# Autodesk Inventor assembly: whole car
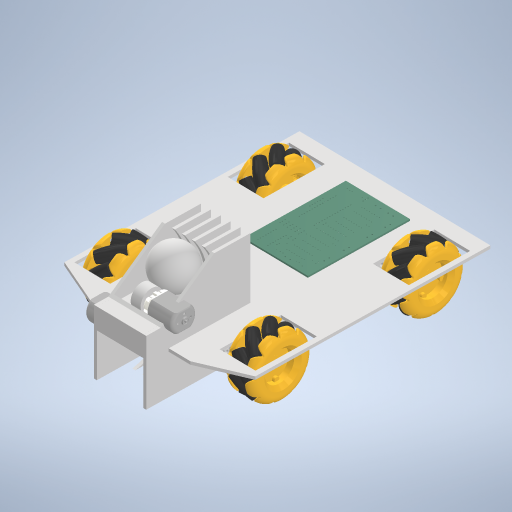
[picture p0: Inventor's stored thumbnail of the model, 512x512]
Saved by Autodesk Inventor 2023.2 (Build 272271030, 271C)
## iProperties
Created: 2023-06-19
Part Number: whole car
Document SubType Name: Assembly
Designer: kao91
Author: kao91
## Documents named in this file (16)
- C:\Users\kao91\Desktop\github\NTNU_mechatronic_practice_project\car design\whole car.iam
- C:\Users\kao91\Desktop\github\NTNU_mechatronic_practice_project\car design\DC Motor Gearbox\DC Motor Gearbox.ipt
- C:\Users\kao91\Desktop\github\NTNU_mechatronic_practice_project\car design\DC Motor Gearbox\DC Motor Gearbox_MIR.ipt
- C:\Users\kao91\Desktop\github\NTNU_mechatronic_practice_project\car design\df-robot-48mm-mecanum-wheel-left-side-1.snapshot.2\Mecanum Left v5\Mecanum Ra.ipt
- C:\Users\kao91\Desktop\github\NTNU_mechatronic_practice_project\car design\motor_to_mecanum_connector.ipt
- C:\Users\kao91\Desktop\github\NTNU_mechatronic_practice_project\car design\floor.ipt
- C:\Users\kao91\Desktop\github\NTNU_mechatronic_practice_project\car design\car platform.ipt
- C:\Users\kao91\Desktop\github\NTNU_mechatronic_practice_project\car design\df-robot-48mm-mecanum-wheel-left-side-1.snapshot.2\Mecanum Left v5\Mecanum Rb.ipt
- C:\Users\kao91\Desktop\github\NTNU_mechatronic_practice_project\car design\circuitPCB\circuitPCB.ipt
- C:\Users\kao91\Desktop\github\NTNU_mechatronic_practice_project\car design\collectballLR.ipt
- C:\Users\kao91\Desktop\github\NTNU_mechatronic_practice_project\car design\lr.ipt
- C:\Users\kao91\Desktop\github\NTNU_mechatronic_practice_project\car design\PING pong.ipt
- C:\Users\kao91\Desktop\github\NTNU_mechatronic_practice_project\car design\ROTATE.ipt
- C:\Users\kao91\Desktop\github\NTNU_mechatronic_practice_project\car design\FC-280PT-20150 12V DC Motor v3\FC-280PT-20150 12V DC Motor v3.ipt
- C:\Users\kao91\Desktop\github\NTNU_mechatronic_practice_project\car design\roll.ipt
- C:\Users\kao91\Desktop\github\NTNU_mechatronic_practice_project\car design\shoot.ipt
## Components (27 placed, 15 different names)
1. floor:1 — Mate:5, Tangent:5, Mate:23, Mate:24
2. car platform:1 — Flush:9, Mate:6, Mate:8, Mate:11, Mate:12, Mate:13, Mate:14, Mate:15, Mate:16, Flush:17, Flush:18, Flush:19, Flush:20, Mate:17, Flush:21, Mate:18, Mate:19, Mate:20, Mate:21, Mate:22
3. circuitPCB:1 — Mate:6, Flush:19
4. collectballLR:1 — Mate:15, Flush:16, Mate:16
5. collectballLR:2 — Mate:8, Mate:11, Flush:12, Flush:13, Flush:16, Tangent:2
6. collectballLR:3 — Flush:12, Flush:13, Flush:14, Flush:15, Mate:14, Tangent:3
7. collectballLR:4 — Mate:12, Flush:14, Flush:15, Mate:13, Mate:17
8. lr:1 — Flush:21, Mate:18, Mate:19, Tangent:4, Flush:22, Flush:23, Flush:25
9. lr:2 — Mate:20, Mate:21, Mate:22, Flush:24
10. PING pong:1 — Tangent:2, Tangent:3, Tangent:4
11. ROTATE:1 — Flush:22, Mate:25, Flush:23, Flush:24, Flush:27, Flush:28
12. FC-280PT-20150 12V DC Motor v3:1 — Flush:27, Flush:28, Rotational:12
13. FC-280PT-20150 12V DC Motor v3:2 — Mate:25, Flush:25, Flush:26, Rigid:1
14. roll:1 — Flush:26, Rigid:1
15. shoot:1 — Rotational:12
16. DC Motor Gearbox:1 — Rotational:1, Flush:1, Flush:6, Flush:7
17. Mecanum Ra:2 — Rotational:8, Mate:5
18. motor_to_mecanum_connector:1 — Rotational:1, Rotational:8
19. DC Motor Gearbox_MIR:1 — Rotational:4, Flush:2, Flush:5, Flush:7, Flush:17, Flush:20
20. motor_to_mecanum_connector:2 — Rotational:4, Rotational:10, Mate:23
21. Mecanum Rb:2 — Rotational:10
22. DC Motor Gearbox:2 — Rotational:2, Flush:1, Flush:3, Flush:4, Flush:6, Mate:2, Flush:9
23. Mecanum Rb:1 — Rotational:11, Mate:24
24. motor_to_mecanum_connector:4 — Rotational:2, Rotational:11
25. DC Motor Gearbox_MIR:2 — Rotational:3, Flush:2, Flush:3, Flush:4, Flush:5, Mate:2, Flush:18
26. Mecanum Ra:3 — Rotational:9, Tangent:5
27. motor_to_mecanum_connector:3 — Rotational:3, Rotational:9
## Relationships (58: Flush 25, Mate 19, RevoluteJoint 9, Tangent 4, WeldJoint 1)
- Rotational:1 [RevoluteJoint]: DC Motor Gearbox:1 ↔ motor_to_mecanum_connector:1
- Rotational:2 [RevoluteJoint]: DC Motor Gearbox:2 ↔ motor_to_mecanum_connector:4
- Rotational:3 [RevoluteJoint]: DC Motor Gearbox_MIR:2 ↔ motor_to_mecanum_connector:3
- Rotational:4 [RevoluteJoint]: DC Motor Gearbox_MIR:1 ↔ motor_to_mecanum_connector:2
- Rotational:8 [RevoluteJoint]: Mecanum Ra:2 ↔ motor_to_mecanum_connector:1
- Flush:1: DC Motor Gearbox:1 ↔ DC Motor Gearbox:2
- Flush:2: DC Motor Gearbox_MIR:1 ↔ DC Motor Gearbox_MIR:2
- Flush:3: DC Motor Gearbox:2 ↔ DC Motor Gearbox_MIR:2
- Flush:4: DC Motor Gearbox:2 ↔ DC Motor Gearbox_MIR:2
- Flush:5: DC Motor Gearbox_MIR:1 ↔ DC Motor Gearbox_MIR:2
- Flush:6: DC Motor Gearbox:1 ↔ DC Motor Gearbox:2
- Flush:7: DC Motor Gearbox:1 ↔ DC Motor Gearbox_MIR:1
- Mate:2 (-173 mm): DC Motor Gearbox:2 ↔ DC Motor Gearbox_MIR:2
- Mate:5 (30 mm): floor:1 ↔ Mecanum Ra:2
- Flush:9: car platform:1 ↔ DC Motor Gearbox:2
- Rotational:9 [RevoluteJoint]: Mecanum Ra:3 ↔ motor_to_mecanum_connector:3
- Rotational:10 [RevoluteJoint]: motor_to_mecanum_connector:2 ↔ Mecanum Rb:2
- Rotational:11 [RevoluteJoint]: Mecanum Rb:1 ↔ motor_to_mecanum_connector:4
- Mate:6: car platform:1 ↔ circuitPCB:1
- Mate:8: car platform:1 ↔ collectballLR:2
- Mate:11: car platform:1 ↔ collectballLR:2
- Flush:12: collectballLR:2 ↔ collectballLR:3
- Flush:13: collectballLR:2 ↔ collectballLR:3
- Mate:12: car platform:1 ↔ collectballLR:4
- Flush:14: collectballLR:3 ↔ collectballLR:4
- Flush:15: collectballLR:3 ↔ collectballLR:4
- Mate:13: car platform:1 ↔ collectballLR:4
- Mate:14: car platform:1 ↔ collectballLR:3
- Mate:15: car platform:1 ↔ collectballLR:1
- Flush:16: collectballLR:1 ↔ collectballLR:2
- Mate:16: car platform:1 ↔ collectballLR:1
- Flush:17 (-0.5 mm): car platform:1 ↔ DC Motor Gearbox_MIR:1
- Flush:18 (-0.5 mm): car platform:1 ↔ DC Motor Gearbox_MIR:2
- Flush:19 (20 mm): car platform:1 ↔ circuitPCB:1
- Flush:20 (-34 mm): car platform:1 ↔ DC Motor Gearbox_MIR:1
- Mate:17: car platform:1 ↔ collectballLR:4
- Flush:21: car platform:1 ↔ lr:1
- Mate:18: car platform:1 ↔ lr:1
- Mate:19: car platform:1 ↔ lr:1
- Mate:20: car platform:1 ↔ lr:2
- Mate:21: car platform:1 ↔ lr:2
- Mate:22: car platform:1 ↔ lr:2
- Tangent:2: collectballLR:2 ↔ PING pong:1
- Tangent:3: collectballLR:3 ↔ PING pong:1
- Tangent:4: lr:1 ↔ PING pong:1
- Flush:22: lr:1 ↔ ROTATE:1
- Tangent:5: floor:1 ↔ Mecanum Ra:3
- Mate:23 (30 mm): floor:1 ↔ motor_to_mecanum_connector:2
- Mate:24 (30 mm): floor:1 ↔ Mecanum Rb:1
- Mate:25 (-23 mm): ROTATE:1 ↔ FC-280PT-20150 12V DC Motor v3:2
- Flush:23: lr:1 ↔ ROTATE:1
- Flush:24: lr:2 ↔ ROTATE:1
- Flush:25 (-18 mm): lr:1 ↔ FC-280PT-20150 12V DC Motor v3:2
- Flush:26: FC-280PT-20150 12V DC Motor v3:2 ↔ roll:1
- Rigid:1 [WeldJoint]: FC-280PT-20150 12V DC Motor v3:2 ↔ roll:1
- Flush:27 (-13 mm): ROTATE:1 ↔ FC-280PT-20150 12V DC Motor v3:1
- Flush:28 (-12 mm): ROTATE:1 ↔ FC-280PT-20150 12V DC Motor v3:1
- Rotational:12 [RevoluteJoint]: FC-280PT-20150 12V DC Motor v3:1 ↔ shoot:1
